# Autodesk Inventor assembly: Dropdown_Assembly_V3_Complete
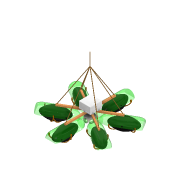
[picture p0: Inventor's stored thumbnail of the model, 180x180]
Saved by Autodesk Inventor 2021 (Build 250183000, 183)
## iProperties
Created: 2020-07-21
Part Number: Dropdown_Assembly_V3_Complete
Document SubType Name: Assembly
Designer: cameron
Mass: 983.451 g
Surface Area: 13621.7 cm^2
Volume: 1178.19 cm^3
Density: 0.834714 g/cm^3
Author: cameron
## Documents named in this file (7)
- C:\Users\camer\Git\Sure2020-DropdownSystem\InventorDropsonde\Dropdown_Assembly_V3_Complete.iam
- C:\Users\camer\Git\Sure2020-DropdownSystem\InventorDropsonde\PVC center piece.ipt
- C:\Users\camer\Git\Sure2020-DropdownSystem\InventorDropsonde\Dropdown_Assembly_V3.iam
- C:\Users\camer\Git\Sure2020-DropdownSystem\InventorDropsonde\Top rods.ipt
- C:\Users\camer\Git\Sure2020-DropdownSystem\InventorDropsonde\PCB housing.ipt
- C:\Users\camer\Git\Sure2020-DropdownSystem\InventorDropsonde\C brace.ipt
- C:\Users\camer\Git\Sure2020-DropdownSystem\InventorDropsonde\Balloon_Rope.ipt
## Components (16 placed, 6 different names)
1. PVC center piece:1 — Mate:1, Mate:2
2. Top rods:1 — Tangent:1, Tangent:2, Mate:3, Mate:4, Mate:6, Mate:8, Mate:10, Mate:12, Mate:14, Flush:1, Flush:2
3. PCB housing:1 — Mate:3, Mate:5, Mate:7, Mate:9, Mate:11, Mate:13, Mate:15
4. C brace:1 — Mate:10, Mate:11
5. C brace:2 — Mate:12, Mate:13
6. C brace:3 — Mate:4, Mate:5
7. C brace:4 — Mate:6, Mate:7
8. C brace:5 — Mate:8, Mate:9
9. C brace:6 — Mate:14, Mate:15
10. Balloon_Rope:1 — Flush:2, Flush:3
11. Dropdown_Assembly_V3:1 [sub-assembly] — Mate:1, Mate:2
12. Dropdown_Assembly_V3:2 [sub-assembly] — Tangent:2
13. Dropdown_Assembly_V3:3 [sub-assembly]
14. Dropdown_Assembly_V3:4 [sub-assembly] — Tangent:1
15. Dropdown_Assembly_V3:5 [sub-assembly]
16. Dropdown_Assembly_V3:6 [sub-assembly]
## Component patterns: (6 elements, first: Dropdown_Assembly_V3:1)
## Relationships (20: Mate 15, Flush 3, Tangent 2)
- Mate:1: PVC center piece:1 ↔ Dropdown_Assembly_V3:1
- Mate:2: PVC center piece:1 ↔ Dropdown_Assembly_V3:1
- Tangent:1: Top rods:1 ↔ Dropdown_Assembly_V3:4
- Tangent:2: Top rods:1 ↔ Dropdown_Assembly_V3:2
- Mate:3 (1 mm): Top rods:1 ↔ PCB housing:1
- Mate:4: Top rods:1 ↔ C brace:3
- Mate:5: PCB housing:1 ↔ C brace:3
- Mate:6: Top rods:1 ↔ C brace:4
- Mate:7: PCB housing:1 ↔ C brace:4
- Mate:8: Top rods:1 ↔ C brace:5
- Mate:9: PCB housing:1 ↔ C brace:5
- Mate:10: Top rods:1 ↔ C brace:1
- Mate:11: PCB housing:1 ↔ C brace:1
- Mate:12: Top rods:1 ↔ C brace:2
- Mate:13: PCB housing:1 ↔ C brace:2
- Mate:14: Top rods:1 ↔ C brace:6
- Mate:15: PCB housing:1 ↔ C brace:6
- Flush:1 (300 mm): Top rods:1
- Flush:2: Top rods:1 ↔ Balloon_Rope:1
- Flush:3: Balloon_Rope:1
